# Autodesk Inventor assembly: 12 Geneva Assembly
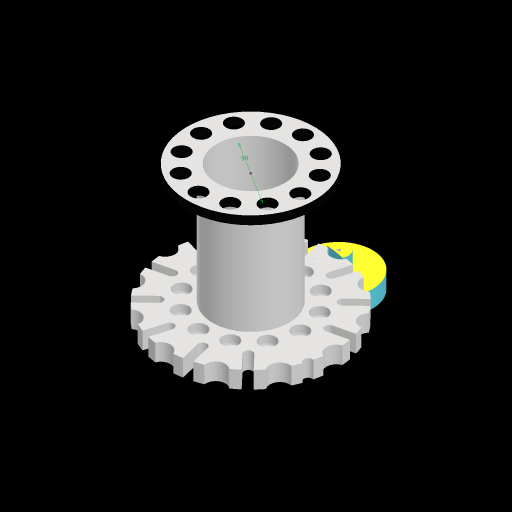
[picture p0: Inventor's stored thumbnail of the model, 512x512]
Saved by Autodesk Inventor 2023 (Build 270158000, 158)
## iProperties
Created: 2022-10-22
Part Number: 12 Geneva Assembly
Document SubType Name: Assembly
Designer: annah
Author: annah
## Documents named in this file (5)
- C:\Users\annah\Documents\GitHub\BehrendURCMechanical\CAD\Science\12 Geneva Assembly.iam
- C:\Users\annah\Documents\GitHub\BehrendURCMechanical\CAD\Science\Bridge 12.ipt
- C:\Users\annah\Documents\GitHub\BehrendURCMechanical\CAD\Science\Geneva Circle arc 12.ipt
- C:\Users\annah\Documents\GitHub\BehrendURCMechanical\CAD\Science\Geneva Gear 12.ipt
- C:\Users\annah\Documents\GitHub\BehrendURCMechanical\CAD\Science\12 Test Tube Rack.ipt
## Components (4 placed, 4 different names)
1. Bridge 12:1 — Mate:1, Mate:2, Mate:3, Mate:4, Mate:5, Mate:8
2. Geneva Circle arc 12:1 — Mate:2, Mate:3
3. Geneva Gear 12:1 — Mate:4, Mate:5, Mate:6, Mate:7
4. 12 Test Tube Rack:1 — Mate:6, Mate:7, Mate:8
## Relationships (8: Mate 8)
- Mate:1: Bridge 12:1
- Mate:2: Bridge 12:1 ↔ Geneva Circle arc 12:1
- Mate:3: Bridge 12:1 ↔ Geneva Circle arc 12:1
- Mate:4: Bridge 12:1 ↔ Geneva Gear 12:1
- Mate:5: Bridge 12:1 ↔ Geneva Gear 12:1
- Mate:6: Geneva Gear 12:1 ↔ 12 Test Tube Rack:1
- Mate:7: Geneva Gear 12:1 ↔ 12 Test Tube Rack:1
- Mate:8: Bridge 12:1 ↔ 12 Test Tube Rack:1
